# Autodesk Inventor assembly: full-model
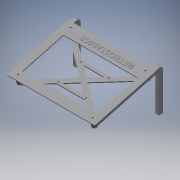
[picture p0: Inventor's stored thumbnail of the model, 180x180]
Saved by Autodesk Inventor 2018 (Build 220112000, 112)
## iProperties
Created: 2017-11-15
Part Number: full-model
Document SubType Name: Assembly
Designer: WutchZone
Author: WutchZone
## Documents named in this file (5)
- D:\Meteostanice\full-model.iam
- D:\Meteostanice\LCD-holder-left.ipt
- D:\Meteostanice\LCD-holder-right.ipt
- D:\Meteostanice\LCD-backcover.ipt
- D:\Meteostanice\LCD-frontcover.ipt
## Components (4 placed, 4 different names)
1. LCD-holder-left — Mate:2, Mate:3, Mate:6, Mate:7, Mate:8
2. LCD-holder-right:1 — Mate:1, Mate:4, Mate:5, Mate:9, Mate:10
3. LCD-backcover:1 — Mate:3, Mate:5, Mate:6
4. LCD-frontcover:1 — Mate:1, Mate:2, Mate:4, Mate:7, Mate:8
## Relationships (10: Mate 10)
- Mate:1: LCD-holder-right:1 ↔ LCD-frontcover:1
- Mate:2: LCD-holder-left ↔ LCD-frontcover:1
- Mate:3: LCD-holder-left ↔ LCD-backcover:1
- Mate:4: LCD-holder-right:1 ↔ LCD-frontcover:1
- Mate:5: LCD-holder-right:1 ↔ LCD-backcover:1
- Mate:6: LCD-holder-left ↔ LCD-backcover:1
- Mate:7: LCD-holder-left ↔ LCD-frontcover:1
- Mate:8: LCD-holder-left ↔ LCD-frontcover:1
- Mate:9: LCD-holder-right:1
- Mate:10: LCD-holder-right:1
